# Autodesk Inventor assembly: BackLink
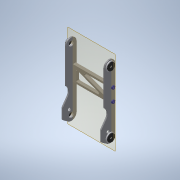
[picture p0: Inventor's stored thumbnail of the model, 180x180]
Saved by Autodesk Inventor 2022.4 (Build 264492000, 492)
## iProperties
Created: 2016-08-23
Part Number: BackLink
Material: 一般
Document SubType Name: Assembly
Designer: hiro
Mass: 29.252 g
Surface Area: 149.463 cm^2
Volume: 12.3578 cm^3
Density: 2.3671 g/cm^3
Author: hiro
## Documents named in this file (6)
- C:\Users\supra\Documents\GitHub\OpenPlatform_ver3_0\LowerBody\Link\BackLink.iam
- C:\Users\supra\Documents\GitHub\OpenPlatform_ver3_0\LowerBody\Link\BackLink_diagonal.ipt
- C:\Users\supra\Documents\GitHub\OpenPlatform_ver3_0\Ready_Made\UUW-0312-10BH.ipt
- C:\Users\supra\Documents\GitHub\OpenPlatform_ver3_0\Ready_Made\Screw\M3-6.ipt
- C:\Users\supra\Documents\GitHub\OpenPlatform_ver3_0\LowerBody\Link\BackLink_frame.ipt
- C:\Users\supra\Documents\GitHub\OpenPlatform_ver3_0\Ready_Made\TT-0814-15.ipt
## Components (15 placed, 5 different names)
1. UUW-0312-10BH:1 — 挿入:49
2. UUW-0312-10BH:2 — 挿入:46
3. UUW-0312-10BH:3 — 挿入:47
4. UUW-0312-10BH:4 — 挿入:48
5. BackLink_diagonal:1 — 挿入:31, 挿入:32, 挿入:33, 挿入:34, フラッシュ:1, メイト:1
6. M3-6:1 — 挿入:38
7. M3-6:2 — 挿入:37
8. M3-6:3 — 挿入:41
9. M3-6:4 — 挿入:40
10. BackLink_frame:1 — 挿入:33, 挿入:34, 挿入:37, 挿入:38, 挿入:42, 挿入:45
11. BackLink_frame:2 — 挿入:31, 挿入:32, 挿入:40, 挿入:41, フラッシュ:2, 挿入:43, 挿入:44
12. TT-0814-15:1 — 挿入:42, 挿入:47
13. TT-0814-15:2 — 挿入:43, 挿入:48
14. TT-0814-15:3 — 挿入:44, 挿入:49
15. TT-0814-15:4 — 挿入:45, 挿入:46
## Relationships (19: Insert 16, Flush 2, Mate 1)
- 挿入:31 [Insert]: BackLink_diagonal:1 ↔ BackLink_frame:2
- 挿入:32 [Insert]: BackLink_diagonal:1 ↔ BackLink_frame:2
- 挿入:33 [Insert]: BackLink_diagonal:1 ↔ BackLink_frame:1
- 挿入:34 [Insert]: BackLink_diagonal:1 ↔ BackLink_frame:1
- 挿入:37 [Insert]: M3-6:2 ↔ BackLink_frame:1
- 挿入:38 [Insert]: M3-6:1 ↔ BackLink_frame:1
- 挿入:40 [Insert]: M3-6:4 ↔ BackLink_frame:2
- 挿入:41 [Insert]: M3-6:3 ↔ BackLink_frame:2
- フラッシュ:1 [Flush]: BackLink_diagonal:1
- メイト:1 [Mate]: BackLink_diagonal:1
- フラッシュ:2 [Flush]: BackLink_frame:2
- 挿入:42 [Insert]: BackLink_frame:1 ↔ TT-0814-15:1
- 挿入:43 [Insert]: BackLink_frame:2 ↔ TT-0814-15:2
- 挿入:44 [Insert]: BackLink_frame:2 ↔ TT-0814-15:3
- 挿入:45 [Insert]: BackLink_frame:1 ↔ TT-0814-15:4
- 挿入:46 [Insert]: UUW-0312-10BH:2 ↔ TT-0814-15:4
- 挿入:47 [Insert]: UUW-0312-10BH:3 ↔ TT-0814-15:1
- 挿入:48 [Insert]: UUW-0312-10BH:4 ↔ TT-0814-15:2
- 挿入:49 [Insert]: UUW-0312-10BH:1 ↔ TT-0814-15:3
